# Autodesk Inventor assembly: bogie
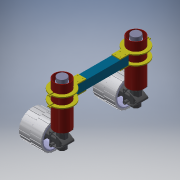
[picture p0: Inventor's stored thumbnail of the model, 180x180]
Saved by Autodesk Inventor 2018 (Build 220112000, 112)
## iProperties
Created: 2017-10-24
Part Number: bogie
Material: 一般
Document SubType Name: Assembly
Designer: 翔
Author: 翔
## Documents named in this file (4)
- E:\forest_robot_cad\Forest_v4\bogie.iam
- E:\forest_robot_cad\Forest_v4\wheel\motor_set01.iam
- E:\forest_robot_cad\Forest_v4\wheel\motor_hold_sample.ipt
- E:\forest_robot_cad\Forest_v4\bogie_bar_sample_300.ipt
## Components (7 placed, 3 different names)
1. motor_set01:1 [sub-assembly] — メイト:1, メイト:2, フラッシュ:3, フラッシュ:6
2. motor_set01:2 [sub-assembly] — メイト:3, メイト:4, フラッシュ:4, フラッシュ:5, フラッシュ:6
3. motor_hold_sample:1 — メイト:1, メイト:5, メイト:6, メイト:7, フラッシュ:3
4. motor_hold_sample:2 — メイト:2, メイト:8, メイト:9, メイト:10
5. motor_hold_sample:3 — メイト:3, フラッシュ:4, メイト:11, メイト:12, メイト:13
6. motor_hold_sample:4 — メイト:4, メイト:14, メイト:15, メイト:16
7. bogie_bar_sample_300:1 — フラッシュ:1, フラッシュ:2, メイト:5, メイト:6, メイト:7, メイト:8, メイト:9, メイト:10, メイト:11, メイト:12, メイト:13, メイト:14, メイト:15, メイト:16, フラッシュ:5
## Relationships (22: Mate 16, Flush 6)
- メイト:1 [Mate]: motor_set01:1 ↔ motor_hold_sample:1
- メイト:2 [Mate]: motor_set01:1 ↔ motor_hold_sample:2
- メイト:3 [Mate]: motor_set01:2 ↔ motor_hold_sample:3
- メイト:4 [Mate]: motor_set01:2 ↔ motor_hold_sample:4
- フラッシュ:1 [Flush]: bogie_bar_sample_300:1
- フラッシュ:2 [Flush]: bogie_bar_sample_300:1
- メイト:5 [Mate]: motor_hold_sample:1 ↔ bogie_bar_sample_300:1
- メイト:6 [Mate]: motor_hold_sample:1 ↔ bogie_bar_sample_300:1
- メイト:7 [Mate]: motor_hold_sample:1 ↔ bogie_bar_sample_300:1
- メイト:8 [Mate]: motor_hold_sample:2 ↔ bogie_bar_sample_300:1
- メイト:9 [Mate]: motor_hold_sample:2 ↔ bogie_bar_sample_300:1
- メイト:10 [Mate]: motor_hold_sample:2 ↔ bogie_bar_sample_300:1
- フラッシュ:3 [Flush] (50 mm): motor_set01:1 ↔ motor_hold_sample:1
- フラッシュ:4 [Flush] (-50 mm): motor_set01:2 ↔ motor_hold_sample:3
- メイト:11 [Mate]: motor_hold_sample:3 ↔ bogie_bar_sample_300:1
- メイト:12 [Mate]: motor_hold_sample:3 ↔ bogie_bar_sample_300:1
- メイト:13 [Mate]: motor_hold_sample:3 ↔ bogie_bar_sample_300:1
- メイト:14 [Mate]: motor_hold_sample:4 ↔ bogie_bar_sample_300:1
- メイト:15 [Mate]: motor_hold_sample:4 ↔ bogie_bar_sample_300:1
- メイト:16 [Mate]: motor_hold_sample:4 ↔ bogie_bar_sample_300:1
- フラッシュ:5 [Flush] (149.5 mm): motor_set01:2 ↔ bogie_bar_sample_300:1
- フラッシュ:6 [Flush]: motor_set01:1 ↔ motor_set01:2
